# Autodesk Inventor assembly: noseAssembly
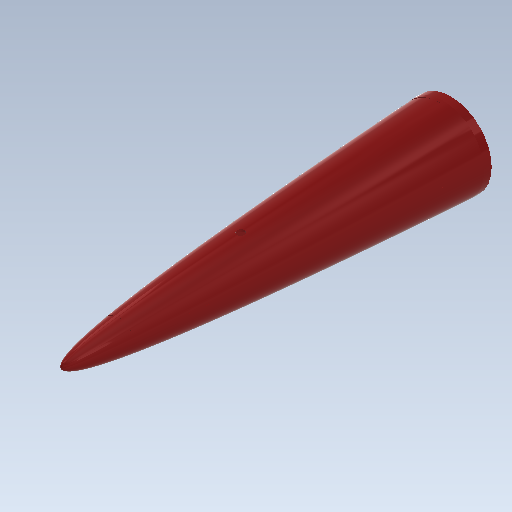
[picture p0: Inventor's stored thumbnail of the model, 512x512]
Saved by Autodesk Inventor 2020.3 (Build 243373000, 373)
## iProperties
Created: 2021-03-12
Part Number: noseAssembly
Document SubType Name: Assembly
Designer: 0x6f736f646f
Author: 0x6f736f646f
## Documents named in this file (3)
- C:\Users\0x6f736f646f\OneDrive\Documents\Nakuja\airframev1\Design\noseAssembly.iam
- C:\Users\0x6f736f646f\OneDrive\Documents\Nakuja\airframev1\Design\nose-basepart1.ipt
- C:\Users\0x6f736f646f\OneDrive\Documents\Nakuja\airframev1\Design\nose-toppart1.ipt
## Components (2 placed, 2 different names)
1. nose-basepart1:1 — Flush:1, Flush:2, Mate:1
2. nose-toppart1:1 — Flush:1, Flush:2, Mate:1
## Relationships (3: Flush 2, Mate 1)
- Flush:1: nose-basepart1:1 ↔ nose-toppart1:1
- Flush:2: nose-basepart1:1 ↔ nose-toppart1:1
- Mate:1: nose-basepart1:1 ↔ nose-toppart1:1
